# Autodesk Inventor assembly: ASY GNH 011 Dilution point Frame1
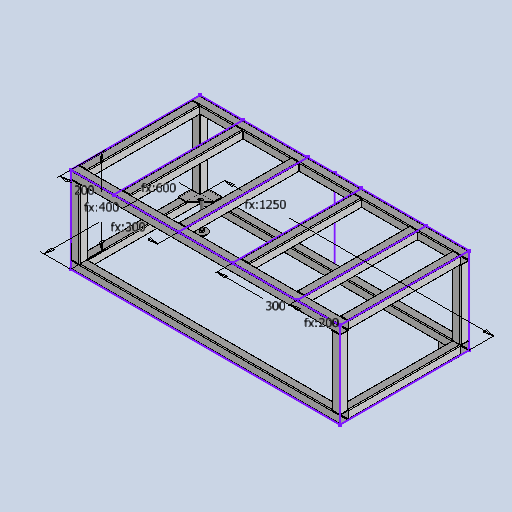
[picture p0: Inventor's stored thumbnail of the model, 512x512]
Saved by Autodesk Inventor 2025.1 (Build 291241020, 241B)
## iProperties
Created: 2025-03-06
Part Number: ASY GNH 011 Dilution point Frame1
Document SubType Name: Assembly
Designer: user
_SolveAssemblyDoc: Frame Generator Solve Assembly
_Version: 25.0.0
Author: user
## Documents named in this file (6)
- C:\Users\user\YandexDisk-badmisterfox\home pc\Inventor\GNH-Petrodvorec\ASY GNH 010 Dilution point Frame.iam
- C:\Users\user\YandexDisk-badmisterfox\home pc\Inventor\GNH-Petrodvorec\GNH 010 frame.ipt
- C:\Users\user\YandexDisk-badmisterfox\home pc\Inventor\GNH-Petrodvorec\ASY GNH 010 Dilution point Frame\Frame\Frame 1741245058463.iam
- C:\Users\user\YandexDisk-badmisterfox\home pc\Inventor\GNH-Petrodvorec\GNH 015 leg support.ipt
- C:\Users\user\YandexDisk-badmisterfox\home pc\Inventor\GNH-Petrodvorec\Content Center Files\en-US\ISO 8676(1)\ISO 8676 - M12 x 1.25 x 120DIN EN.ipt
- C:\Users\user\YandexDisk-badmisterfox\home pc\Inventor\GNH-Petrodvorec\GNH 015 leg plate.ipt
## Components (6 placed, 5 different names)
1. GNH 011 Dilution frame sketch:1
2. Frame 1741245058463:1 [sub-assembly] — Mate:1, Flush:1, Flush:2, Mate:2, Flush:3, Flush:4
3. GNH 081 leg support:1 — Mate:1, Flush:1, Flush:2
4. ISO 8676 - M12 x 1.25 x 120:1 — Rigid:2
5. GNH 082 leg plate:1 — Rigid:2
6. GNH 081 leg support:2 — Mate:2, Flush:3, Flush:4
## Relationships (7: Flush 4, Mate 2, WeldJoint 1)
- Mate:1: Frame 1741245058463:1 ↔ GNH 081 leg support:1
- Flush:1: Frame 1741245058463:1 ↔ GNH 081 leg support:1
- Flush:2: Frame 1741245058463:1 ↔ GNH 081 leg support:1
- Rigid:2 [WeldJoint]: ISO 8676 - M12 x 1.25 x 120:1 ↔ GNH 082 leg plate:1
- Mate:2: Frame 1741245058463:1 ↔ GNH 081 leg support:2
- Flush:3: Frame 1741245058463:1 ↔ GNH 081 leg support:2
- Flush:4: Frame 1741245058463:1 ↔ GNH 081 leg support:2
